# Autodesk Inventor assembly: 7
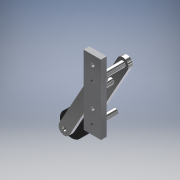
[picture p0: Inventor's stored thumbnail of the model, 180x180]
Saved by Autodesk Inventor 2019 (Build 230136000, 136)
## iProperties
Created: 2018-11-14
Part Number: 7
Document SubType Name: Assembly
Designer: steelen
Description: Spring Chain Tensioner
Material_size: As Specified
Quantity: 2
Author: steelen
## Documents named in this file (7)
- P:\me_fsae\2018_2019\ME\DriveTrain\SpringTensioner\TensionerASM.iam
- P:\me_fsae\2018_2019\ME\DriveTrain\SpringTensioner\TensionerBase.ipt
- P:\me_fsae\2018_2019\ME\DriveTrain\SpringTensioner\TensionerBar.ipt
- P:\me_fsae\2018_2019\ME\DriveTrain\SpringTensioner\RollerBar.ipt
- P:\me_fsae\2018_2019\ME\DriveTrain\SpringTensioner\SpringBar2.ipt
- P:\me_fsae\2018_2019\ME\DriveTrain\SpringTensioner\PivotBar.ipt
- P:\me_fsae\2018_2019\ME\DriveTrain\SpringTensioner\RubberRoller.ipt
## Components (8 placed, 6 different names)
1. TensionerBase:1 — Mate:1, Mate:2, Mate:3, Insert:1, Insert:2
2. SpringBar2:1 — Insert:1
3. PivotBar:1 — Insert:2, Insert:7
4. TensionerBar:1 — Insert:3, Insert:4, Insert:7
5. RollerBar:1 — Insert:3, Insert:5
6. TensionerBar:3 — Insert:5, Insert:6, Insert:8
7. RollerBar:2 — Insert:4, Insert:6
8. RubberRoller:1 — Insert:8
## Relationships (11: Insert 8, Mate 3)
- Mate:1: TensionerBase:1
- Mate:2: TensionerBase:1
- Mate:3: TensionerBase:1
- Insert:1: TensionerBase:1 ↔ SpringBar2:1
- Insert:2: TensionerBase:1 ↔ PivotBar:1
- Insert:3: TensionerBar:1 ↔ RollerBar:1
- Insert:4: TensionerBar:1 ↔ RollerBar:2
- Insert:5: RollerBar:1 ↔ TensionerBar:3
- Insert:6: TensionerBar:3 ↔ RollerBar:2
- Insert:7: PivotBar:1 ↔ TensionerBar:1
- Insert:8: TensionerBar:3 ↔ RubberRoller:1
